# Autodesk Inventor assembly: Anglerfish_opticsmodule_v0
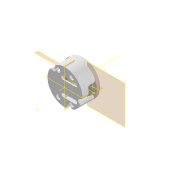
[picture p0: Inventor's stored thumbnail of the model, 180x180]
Saved by Autodesk Inventor 2022 (Build 260153000, 153)
## iProperties
Created: 2022-04-19
Part Number: Anglerfish_opticsmodule_v0
Document SubType Name: Assembly
Designer: Prakash Lab
Author: Prakash Lab
## Documents named in this file (6)
- C:\Users\PrakashLab\Documents\Matchboxscope\INVENTOR\Anglerfish_opticsmodule_v0.iam
- C:\Users\PrakashLab\Documents\Matchboxscope\INVENTOR\Matchboxscope_middle2_v1.ipt
- C:\Users\PrakashLab\Documents\Matchboxscope\INVENTOR\Matchboxscope_bottom_v0.ipt
- C:\Users\PrakashLab\Documents\Matchboxscope\INVENTOR\00_ESP3-CAM.iam
- C:\Users\PrakashLab\Documents\Matchboxscope\INVENTOR\Anglerfish_3inch_tube_adapterplate_focus.ipt
- C:\Users\PrakashLab\Documents\Matchboxscope\INVENTOR\Matchboxscope_lenstube_v0.ipt
## Components (5 placed, 5 different names)
1. 00_ESP3-CAM:1 [sub-assembly]
2. Matchboxscope_middle2_v1:1 — Mate:4, Mate:5
3. Matchboxscope_lenstube_v0:1 — Mate:3
4. Matchboxscope_bottom_v0:1
5. Anglerfish_3inch_tube_adapterplate_focus:1 — Mate:3, Mate:4, Mate:5
## Relationships (8: Mate 5, Insert 2, Flush 1)
- [Mate]: 00_ESP3-CAM:1 ↔ Matchboxscope_bottom_v0:1
- [Flush]: 00_ESP3-CAM:1 ↔ Matchboxscope_bottom_v0:1
- [Insert]: 00_ESP3-CAM:1 ↔ Matchboxscope_middle2_v1:1
- [Mate]: Matchboxscope_middle2_v1:1 ↔ Matchboxscope_bottom_v0:1
- [Insert]: Matchboxscope_middle2_v1:1 ↔ Matchboxscope_lenstube_v0:1
- Mate:3: Matchboxscope_lenstube_v0:1 ↔ Anglerfish_3inch_tube_adapterplate_focus:1
- Mate:4: Matchboxscope_middle2_v1:1 ↔ Anglerfish_3inch_tube_adapterplate_focus:1
- Mate:5 (5 mm): Matchboxscope_middle2_v1:1 ↔ Anglerfish_3inch_tube_adapterplate_focus:1
## Named parameters: d3_d14 = 0 mm, d3_d8 = 0 mm
